# Autodesk Inventor assembly: stepperMotorAndMount
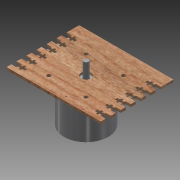
[picture p0: Inventor's stored thumbnail of the model, 180x180]
Saved by Autodesk Inventor 2013 (Build 170138000, 138)
## iProperties
Created: 2013-02-24
Part Number: stepperMotorAndMount
Document SubType Name: Assembly
Designer: Nano
Author: Nano
## Documents named in this file (4)
- C:\Users\Nano\Documents\InventorByron\InventorMasterProject\gyroPhone01\stepperMotorAndMount.iam
- C:\Users\Nano\Documents\InventorByron\InventorMasterProject\gyroPhone01\gearAssemblyTake02\stepperMotorMountPlate01.ipt
- C:\Users\Nano\Documents\InventorByron\InventorMasterProject\gyroPhone01\stepperMotorBody.ipt
- C:\Users\Nano\Documents\InventorByron\InventorMasterProject\gyroPhone01\stepperMotorAxel.ipt
## Components (3 placed, 3 different names)
1. stepperMotorMountPlate01:1 — Mate:1, Mate:2, Mate:3
2. stepperMotorBody:1 — Flush:1, Mate:1, Mate:2, Mate:3, Flush:2, Flush:3
3. stepperMotorAxel:1 — Flush:2, Flush:3
## Relationships (6: Flush 3, Mate 3)
- Flush:1: stepperMotorBody:1
- Mate:1: stepperMotorMountPlate01:1 ↔ stepperMotorBody:1
- Mate:2: stepperMotorMountPlate01:1 ↔ stepperMotorBody:1
- Mate:3: stepperMotorMountPlate01:1 ↔ stepperMotorBody:1
- Flush:2: stepperMotorBody:1 ↔ stepperMotorAxel:1
- Flush:3: stepperMotorBody:1 ↔ stepperMotorAxel:1
